# Autodesk Inventor assembly: 276-2168
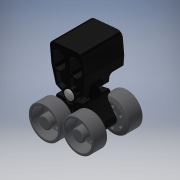
[picture p0: Inventor's stored thumbnail of the model, 180x180]
Saved by Autodesk Inventor 2019.4 (Build 234330000, 330)
## iProperties
Category: Motion
Company: Autodesk Inc.
Created: 2012-04-10
Part Number: 276-2168
Document SubType Name: Assembly
Designer: Autodesk Inc.
Catalog Web Link: http://www.vexrobotics.com/276-2168.html
Vendor: VEX
Author: Autodesk Inc.
## Documents named in this file (6)
- D:\2019-2020TowerTakeOverCad\ncrCadLib\链轮履带\Tank Drive Idler Double Wheel.iam
- D:\2019-2020TowerTakeOverCad\ncrCadLib\链轮履带\零件\IDLER-WHEEL-ROLLER.ipt
- D:\2019-2020TowerTakeOverCad\ncrCadLib\链轮履带\零件\IDLER-DOUBLE-WHEEL-SUPPORT-BOT.ipt
- D:\2019-2020TowerTakeOverCad\ncrCadLib\链轮履带\零件\IDLER-WHEEL-AXLE.ipt
- D:\2019-2020TowerTakeOverCad\ncrCadLib\链轮履带\零件\IDLER-DOUBLE-WHEEL-RIVET.ipt
- D:\2019-2020TowerTakeOverCad\ncrCadLib\链轮履带\零件\IDLER-DOUBLE-WHEEL-SUPPORT-TOP.ipt
## Components (9 placed, 5 different names)
1. IDLER-WHEEL-ROLLER — Insert:4
2. IDLER-DOUBLE-WHEEL-SUPPORT-BOT — Insert:1, Mate:1, Mate:2, Mate:3, Mate:4
3. IDLER-WHEEL-AXLE — Mate:2, Insert:4, Insert:5
4. IDLER-WHEEL-ROLLER — Insert:6, Mate:3
5. IDLER-WHEEL-AXLE — Mate:1, Insert:3, Insert:6
6. IDLER-WHEEL-ROLLER — Insert:5, Mate:4
7. IDLER-DOUBLE-WHEEL-RIVET — Insert:2
8. IDLER-DOUBLE-WHEEL-SUPPORT-TOP — Insert:1, Insert:2
9. IDLER-WHEEL-ROLLER — Insert:3
## Relationships (10: Insert 6, Mate 4)
- Insert:1: IDLER-DOUBLE-WHEEL-SUPPORT-BOT ↔ IDLER-DOUBLE-WHEEL-SUPPORT-TOP
- Insert:2: IDLER-DOUBLE-WHEEL-RIVET ↔ IDLER-DOUBLE-WHEEL-SUPPORT-TOP
- Mate:1: IDLER-DOUBLE-WHEEL-SUPPORT-BOT ↔ IDLER-WHEEL-AXLE
- Mate:2: IDLER-DOUBLE-WHEEL-SUPPORT-BOT ↔ IDLER-WHEEL-AXLE
- Insert:3: IDLER-WHEEL-AXLE ↔ IDLER-WHEEL-ROLLER
- Insert:4: IDLER-WHEEL-ROLLER ↔ IDLER-WHEEL-AXLE
- Insert:5: IDLER-WHEEL-AXLE ↔ IDLER-WHEEL-ROLLER
- Insert:6: IDLER-WHEEL-ROLLER ↔ IDLER-WHEEL-AXLE
- Mate:3: IDLER-DOUBLE-WHEEL-SUPPORT-BOT ↔ IDLER-WHEEL-ROLLER
- Mate:4: IDLER-DOUBLE-WHEEL-SUPPORT-BOT ↔ IDLER-WHEEL-ROLLER
